# Autodesk Inventor assembly: Assembled
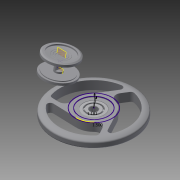
[picture p0: Inventor's stored thumbnail of the model, 180x180]
Saved by Autodesk Inventor 2018 (Build 220112000, 112)
## iProperties
Created: 2017-12-13
Part Number: Assembled
Document SubType Name: Assembly
Designer: Rus
Author: Rus
## Documents named in this file (4)
- E:\Libraries\Documents\3D Models\Spinners and Tops\Circles\Assembled2.iam
- E:\Libraries\Documents\3D Models\Spinners and Tops\Circles\608-bearing2.ipt
- E:\Libraries\Documents\3D Models\Spinners and Tops\Circles\Spinner 2.ipt
- E:\Libraries\Documents\3D Models\Spinners and Tops\Circles\Caps 8mm Square Rounded Caps Male2.ipt
## Components (4 placed, 3 different names)
1. 608-bearing2:1 — Insert:1
2. Spinner 2:1 — Insert:1
3. Caps 8mm Square Rounded Caps Male2:1 — Mate:1, Angle:1, Tangent:1
4. Caps 8mm Square Rounded Caps Male2:2 — Mate:1, Angle:1, Tangent:1
## Relationships (4: Insert 1, Mate 1, Angle 1, Tangent 1)
- Insert:1: 608-bearing2:1 ↔ Spinner 2:1
- Mate:1: Caps 8mm Square Rounded Caps Male2:1 ↔ Caps 8mm Square Rounded Caps Male2:2
- Angle:1 (180 deg): Caps 8mm Square Rounded Caps Male2:1 ↔ Caps 8mm Square Rounded Caps Male2:2
- Tangent:1: Caps 8mm Square Rounded Caps Male2:1 ↔ Caps 8mm Square Rounded Caps Male2:2
